# Autodesk Inventor assembly: Odompod
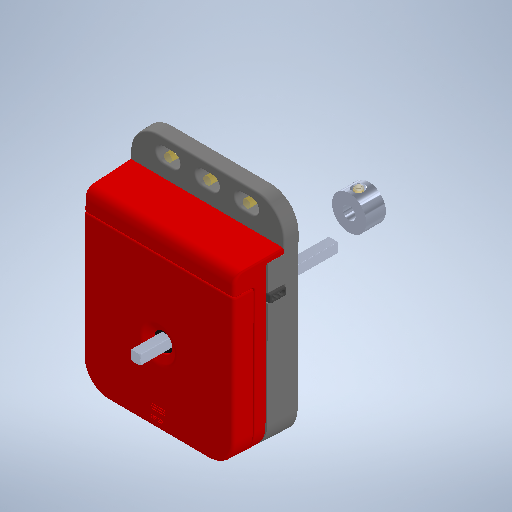
[picture p0: Inventor's stored thumbnail of the model, 512x512]
Saved by Autodesk Inventor 2025.2 (Build 292293000, 293)
## iProperties
Created: 2024-12-19
Part Number: Odompod
Document SubType Name: Assembly
Designer: joshi
Author: joshi
## Documents named in this file (6)
- C:\Users\joshi\Desktop\3388K CAD\Odompod.iam
- C:\Users\joshi\Desktop\3388K CAD\VEX Main\Electronics\Sensors\Optical Shaft Encoder.ipt
- C:\Users\joshi\Desktop\3388K CAD\VEX Main\Motion\Shaft LS\Shaft LS.ipt
- C:\Users\joshi\Desktop\3388K CAD\VEX Main\Motion\Shaft LS\Shaft LS\Shaft LS 2.5.ipt
- C:\Users\joshi\Desktop\3388K CAD\VEX Main\Motion\Shaft LS\Shaft Collar Metal\Shaft Collar No Screw.iam
- C:\Users\joshi\Desktop\3388K CAD\VEX Main\Motion\Shaft LS\Shaft Collar Metal.iam
## Components (3 placed, 3 different names)
1. Optical Shaft Encoder:1 — Mate:1, Mate:2
2. Shaft LS 2.5:1 — Mate:1, Mate:2
3. Shaft Collar No Screw:1 [sub-assembly]
## Relationships (2: Mate 2)
- Mate:1: Optical Shaft Encoder:1 ↔ Shaft LS 2.5:1
- Mate:2: Optical Shaft Encoder:1 ↔ Shaft LS 2.5:1
